# Autodesk Inventor assembly: test fit
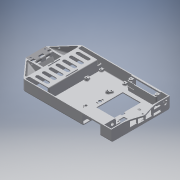
[picture p0: Inventor's stored thumbnail of the model, 180x180]
Saved by Autodesk Inventor 2019 (Build 230136000, 136)
## iProperties
Created: 2020-12-01
Part Number: test fit
Document SubType Name: Assembly
Designer: close
Author: close
## Documents named in this file (3)
- C:\Users\infinity\Documents\GitHub\barc_hardware\Enclosure\Nano&XAVIER\V_2\test fit.iam
- C:\Users\infinity\Documents\GitHub\barc_hardware\Enclosure\Nano&XAVIER\V_2\Enclosure_Dual_v2.ipt
- C:\Users\infinity\Documents\GitHub\barc_hardware\Enclosure\Nano&XAVIER\V_2\hinge_v1.ipt
## Components (2 placed, 2 different names)
1. Enclosure_Dual_v2:1 — Insert:1
2. hinge_v1:1 — Insert:1
## Relationships (1: Insert 1)
- Insert:1 (9.8 mm): Enclosure_Dual_v2:1 ↔ hinge_v1:1
